# Autodesk Inventor assembly: car_2
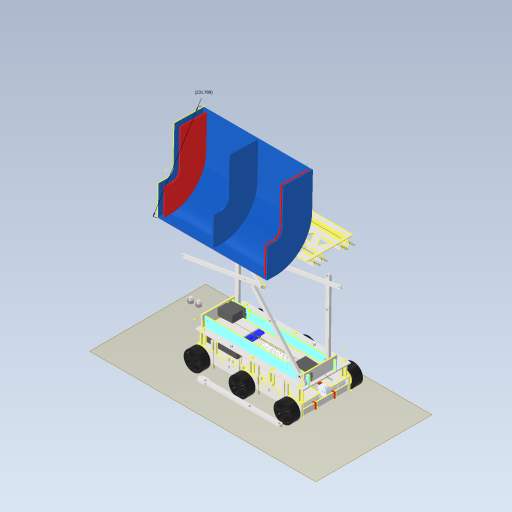
[picture p0: Inventor's stored thumbnail of the model, 512x512]
Saved by Autodesk Inventor 2023 (Build 270158000, 158)
## iProperties
Created: 2023-04-28
Part Number: car_2
Document SubType Name: Assembly
Designer: Johnny Jou
Author: Johnny Jou
## Documents named in this file (19)
- C:\Users\Johnny Jou\Documents\GitHub\Areo_Rider_Cabin\car\car_2.iam
- C:\Users\Johnny Jou\Documents\GitHub\Areo_Rider_Cabin\car\chassis_1_1_3.ipt
- C:\Users\Johnny Jou\Documents\GitHub\Areo_Rider_Cabin\car\外抓檔\25GA370.ipt
- C:\Users\Johnny Jou\Documents\GitHub\Areo_Rider_Cabin\car\chassis_1_5.ipt
- C:\Users\Johnny Jou\Documents\GitHub\Areo_Rider_Cabin\car\chassis_1_6.ipt
- C:\Users\Johnny Jou\Documents\GitHub\Areo_Rider_Cabin\car\plate_2.ipt
- C:\Users\Johnny Jou\Documents\GitHub\Areo_Rider_Cabin\car\bracket.ipt
- C:\Users\Johnny Jou\Documents\GitHub\Areo_Rider_Cabin\car\chassis_1_7.ipt
- C:\Users\Johnny Jou\Documents\GitHub\Areo_Rider_Cabin\car\bearing.ipt
- C:\Users\Johnny Jou\Documents\GitHub\Areo_Rider_Cabin\car\wheel_base_cover.ipt
- C:\Users\Johnny Jou\Documents\GitHub\Areo_Rider_Cabin\car\bracket_2.ipt
- C:\Users\Johnny Jou\Documents\GitHub\Areo_Rider_Cabin\car\外抓檔\BreadBoard.ipt
- C:\Users\Johnny Jou\Documents\GitHub\Areo_Rider_Cabin\car\外抓檔\arduino uno.ipt
- C:\Users\Johnny Jou\Documents\GitHub\Areo_Rider_Cabin\car\外抓檔\L298N.ipt
- C:\Users\Johnny Jou\Documents\GitHub\Areo_Rider_Cabin\car\外抓檔\電池和\3.7V 2X 18650 Battery Holder with On Off Switch_TOP.iam
- C:\Users\Johnny Jou\Documents\GitHub\Areo_Rider_Cabin\car\wheelsys.iam
- C:\Users\Johnny Jou\Documents\GitHub\Areo_Rider_Cabin\Expansion\test\linkage_system_test.iam
- C:\Users\Johnny Jou\Documents\GitHub\Areo_Rider_Cabin\car\axle 4_30.ipt
- C:\Users\Johnny Jou\Documents\GitHub\Areo_Rider_Cabin\Expansion\test\idler.iam
## Components (59 placed, 18 different names)
1. 25GA370:1 — 貼合:7, 貼合:9, 貼合:224
2. 25GA370:2 — 貼合:7, 貼合:8, 貼合:49, 貼合:220
3. chassis_1_5:1 — 貼合:9, 齊平:5, 齊平:10, 齊平:11, 齊平:12, 齊平:13, 貼合:13, 貼合:14, 貼合:42, 貼合:43, 貼合:51
4. chassis_1_5:2 — 貼合:8, 齊平:5, 貼合:15, 貼合:16, 貼合:17, 貼合:18, 貼合:19, 貼合:20
5. chassis_1_6:1 — 齊平:7, 齊平:8, 齊平:9, 齊平:13, 貼合:13, 貼合:14
6. chassis_1_6:2 — 齊平:8, 齊平:10, 貼合:17, 貼合:18, 貼合:42, 貼合:43, 齊平:14, 貼合:44, 貼合:45, 齊平:15
7. chassis_1_6:3 — 齊平:9, 齊平:11, 貼合:19, 貼合:20
8. chassis_1_6:4 — 齊平:7, 齊平:12, 貼合:15, 貼合:16
9. plate_2:1 — 貼合:38, 貼合:40, 貼合:41, 貼合:50, 齊平:19, 貼合:116, 齊平:25, 貼合:185, 貼合:186, 貼合:187, 貼合:188, 貼合:189, 貼合:190, 貼合:191, 貼合:192, 貼合:193, 貼合:194, 貼合:195, 貼合:196, 貼合:197, 貼合:198, 貼合:199, 貼合:200, 貼合:203, 貼合:204, 貼合:205, 貼合:206, 貼合:207, 貼合:208, 貼合:209, 貼合:210, 貼合:211
10. chassis_1_1_3:1 — 齊平:14, 貼合:44, 貼合:45, 貼合:46, 貼合:47, 貼合:48, 貼合:49, 齊平:16, 貼合:108, 貼合:110, 貼合:111, 齊平:24, 貼合:171, 貼合:172, 貼合:217, 貼合:219, 貼合:221
11. chassis_1_1_3:2 — 齊平:15, 齊平:16, 貼合:50, 齊平:19, 貼合:52, 貼合:53, 貼合:54, 貼合:55, 貼合:56, 貼合:57, 貼合:109, 齊平:24, 齊平:25, 貼合:169, 貼合:170, 貼合:223, 貼合:225, 貼合:227, 貼合:230, 貼合:231, 貼合:232, 貼合:233
12. chassis_1_7:1 — 貼合:51, 貼合:52, 貼合:53
13. chassis_1_7:2 — 貼合:54, 貼合:55, 貼合:56, 貼合:57
14. 軸承 GB/T 292-2007 類型 IN - 退回 B724 C:1 — 貼合:67, 貼合:68, 插入:2
15. wheel_base_cover:1 — 貼合:67, 貼合:68, 貼合:171, 貼合:172
16. 軸承 GB/T 292-2007 類型 IN - 退回 B724 C:2 — 插入:3
17. wheel_base_cover:2 — 貼合:108, 貼合:109
18. 軸承 GB/T 292-2007 類型 IN - 退回 B724 C:4 — 插入:1
19. wheel_base_cover:4 — 貼合:110, 貼合:111
20. bracket:10 — 貼合:116, 貼合:210
21. bracket:9 — 貼合:211
22. 軸承 GB/T 292-2007 類型 IN - 退回 B724 C:5 — 插入:4
23. wheel_base_cover:5 — 貼合:169, 貼合:170
24. bracket_2:1 — 貼合:191, 貼合:196, 貼合:197
25. bracket_2:2 — 貼合:188, 貼合:192, 貼合:193
26. bracket_2:3 — 貼合:189, 貼合:194, 貼合:198, 貼合:202
27. bracket_2:4 — 貼合:190, 貼合:195, 貼合:199
28. bracket_2:5 — 貼合:185, 貼合:186, 貼合:187, 貼合:201
29. BreadBoard:1 — 貼合:200, 貼合:201, 貼合:202
30. L298N:1 — 貼合:203, 貼合:208, 貼合:209
31. arduino uno:1 — 貼合:204, 貼合:205, 貼合:206
32. 3.7V 2X 18650 Battery Holder with On Off Switch_TOP:1 [sub-assembly] — 貼合:207
33. wheelsys:1 [sub-assembly] — 貼合:217, 相切:1
34. wheelsys:2 [sub-assembly] — 貼合:220, 貼合:221
35. wheelsys:4 [sub-assembly] — 貼合:219
36. wheelsys:5 [sub-assembly] — 貼合:227
37. wheelsys:6 [sub-assembly] — 貼合:224, 貼合:225
38. wheelsys:7 [sub-assembly] — 貼合:223
39. linkage_system_test:1 [sub-assembly] — 貼合:228, 貼合:229
40. axle 4_30:1 — 插入:1
41. axle 4_30:4 — 插入:4
42. axle 4_30:5 — 插入:3
43. axle 4_30:6 — 插入:2
44. idler:1 [sub-assembly] — 貼合:230, 貼合:231
45. idler:2 [sub-assembly] — 貼合:232, 貼合:233
46. idler:3 [sub-assembly]
47. idler:4 [sub-assembly]
48. bracket:7 — 貼合:38, 貼合:40
49. bracket:8 — 貼合:41
50. bracket:11
51. bracket:12
52. bracket:13
53. bracket:14
54. bracket:15
55. bracket:16
56. bracket:17
57. bracket:18
58. bracket:19 — 貼合:228
59. bracket:20 — 貼合:229
## Component patterns: (6 elements, first: bracket:7 + bracket:8)
## Relationships (114: Mate 94, Flush 14, Insert 4, Angle 1, Tangent 1)
- 貼合:7 [Mate] (20 mm): 25GA370:1 ↔ 25GA370:2
- 貼合:8 [Mate]: 25GA370:2 ↔ chassis_1_5:2
- 貼合:9 [Mate]: 25GA370:1 ↔ chassis_1_5:1
- 齊平:5 [Flush]: chassis_1_5:1 ↔ chassis_1_5:2
- 齊平:7 [Flush]: chassis_1_6:1 ↔ chassis_1_6:4
- 齊平:8 [Flush]: chassis_1_6:1 ↔ chassis_1_6:2
- 齊平:9 [Flush]: chassis_1_6:1 ↔ chassis_1_6:3
- 齊平:10 [Flush]: chassis_1_5:1 ↔ chassis_1_6:2
- 齊平:11 [Flush]: chassis_1_5:1 ↔ chassis_1_6:3
- 齊平:12 [Flush]: chassis_1_5:1 ↔ chassis_1_6:4
- 齊平:13 [Flush]: chassis_1_5:1 ↔ chassis_1_6:1
- 貼合:13 [Mate]: chassis_1_5:1 ↔ chassis_1_6:1
- 貼合:14 [Mate]: chassis_1_5:1 ↔ chassis_1_6:1
- 貼合:15 [Mate]: chassis_1_5:2 ↔ chassis_1_6:4
- 貼合:16 [Mate]: chassis_1_5:2 ↔ chassis_1_6:4
- 貼合:17 [Mate]: chassis_1_5:2 ↔ chassis_1_6:2
- 貼合:18 [Mate]: chassis_1_5:2 ↔ chassis_1_6:2
- 貼合:19 [Mate]: chassis_1_5:2 ↔ chassis_1_6:3
- 貼合:20 [Mate]: chassis_1_5:2 ↔ chassis_1_6:3
- [Mate]: bracket:7 ↔ bracket:8
- [Mate]: bracket:7 ↔ bracket:8
- [Mate]: bracket:7 ↔ bracket:8
- 貼合:38 [Mate]: plate_2:1 ↔ bracket:7
- 貼合:40 [Mate]: plate_2:1 ↔ bracket:7
- 貼合:41 [Mate]: plate_2:1 ↔ bracket:8
- 貼合:42 [Mate]: chassis_1_5:1 ↔ chassis_1_6:2
- 貼合:43 [Mate]: chassis_1_5:1 ↔ chassis_1_6:2
- 齊平:14 [Flush]: chassis_1_6:2 ↔ chassis_1_1_3:1
- 貼合:44 [Mate]: chassis_1_6:2 ↔ chassis_1_1_3:1
- 貼合:45 [Mate]: chassis_1_6:2 ↔ chassis_1_1_3:1
- 貼合:46 [Mate]: chassis_1_1_3:1
- 貼合:47 [Mate]: chassis_1_1_3:1
- 貼合:48 [Mate]: chassis_1_1_3:1
- 貼合:49 [Mate]: 25GA370:2 ↔ chassis_1_1_3:1
- 齊平:15 [Flush]: chassis_1_6:2 ↔ chassis_1_1_3:2
- 齊平:16 [Flush]: chassis_1_1_3:1 ↔ chassis_1_1_3:2
- 貼合:50 [Mate]: plate_2:1 ↔ chassis_1_1_3:2
- 齊平:19 [Flush]: plate_2:1 ↔ chassis_1_1_3:2
- 貼合:51 [Mate]: chassis_1_5:1 ↔ chassis_1_7:1
- 貼合:52 [Mate]: chassis_1_1_3:2 ↔ chassis_1_7:1
- 貼合:53 [Mate]: chassis_1_1_3:2 ↔ chassis_1_7:1
- 貼合:54 [Mate]: chassis_1_1_3:2 ↔ chassis_1_7:2
- 貼合:55 [Mate]: chassis_1_1_3:2 ↔ chassis_1_7:2
- 貼合:56 [Mate]: chassis_1_1_3:2 ↔ chassis_1_7:2
- 貼合:57 [Mate]: chassis_1_1_3:2 ↔ chassis_1_7:2
- 貼合:67 [Mate]: 軸承 GB/T 292-2007 類型 IN - 退回 B724 C:1 ↔ wheel_base_cover:1
- 貼合:68 [Mate]: 軸承 GB/T 292-2007 類型 IN - 退回 B724 C:1 ↔ wheel_base_cover:1
- [Mate]: 軸承 GB/T 292-2007 類型 IN - 退回 B724 C:2 ↔ wheel_base_cover:2
- [Mate]: 軸承 GB/T 292-2007 類型 IN - 退回 B724 C:2 ↔ wheel_base_cover:2
- [Mate]: 軸承 GB/T 292-2007 類型 IN - 退回 B724 C:4 ↔ wheel_base_cover:4
- [Mate]: 軸承 GB/T 292-2007 類型 IN - 退回 B724 C:4 ↔ wheel_base_cover:4
- 貼合:108 [Mate]: chassis_1_1_3:1 ↔ wheel_base_cover:2
- 貼合:109 [Mate]: chassis_1_1_3:2 ↔ wheel_base_cover:2
- 貼合:110 [Mate]: chassis_1_1_3:1 ↔ wheel_base_cover:4
- 貼合:111 [Mate]: chassis_1_1_3:1 ↔ wheel_base_cover:4
- [Mate]: bracket:10 ↔ bracket:9
- [Mate]: bracket:10 ↔ bracket:9
- [Mate]: bracket:10 ↔ bracket:9
- 貼合:116 [Mate]: plate_2:1 ↔ bracket:10
- 齊平:24 [Flush]: chassis_1_1_3:1 ↔ chassis_1_1_3:2
- 齊平:25 [Flush]: plate_2:1 ↔ chassis_1_1_3:2
- [Mate]: 軸承 GB/T 292-2007 類型 IN - 退回 B724 C:5 ↔ wheel_base_cover:5
- [Mate]: 軸承 GB/T 292-2007 類型 IN - 退回 B724 C:5 ↔ wheel_base_cover:5
- 貼合:169 [Mate]: chassis_1_1_3:2 ↔ wheel_base_cover:5
- 貼合:170 [Mate]: chassis_1_1_3:2 ↔ wheel_base_cover:5
- 貼合:171 [Mate]: chassis_1_1_3:1 ↔ wheel_base_cover:1
- 貼合:172 [Mate]: chassis_1_1_3:1 ↔ wheel_base_cover:1
- 貼合:185 [Mate]: plate_2:1 ↔ bracket_2:5
- 貼合:186 [Mate]: plate_2:1 ↔ bracket_2:5
- 貼合:187 [Mate]: plate_2:1 ↔ bracket_2:5
- 貼合:188 [Mate]: plate_2:1 ↔ bracket_2:2
- 貼合:189 [Mate]: plate_2:1 ↔ bracket_2:3
- 貼合:190 [Mate]: plate_2:1 ↔ bracket_2:4
- 貼合:191 [Mate]: plate_2:1 ↔ bracket_2:1
- 貼合:192 [Mate]: plate_2:1 ↔ bracket_2:2
- 貼合:193 [Mate]: plate_2:1 ↔ bracket_2:2
- 貼合:194 [Mate]: plate_2:1 ↔ bracket_2:3
- 貼合:195 [Mate]: plate_2:1 ↔ bracket_2:4
- 貼合:196 [Mate]: plate_2:1 ↔ bracket_2:1
- 貼合:197 [Mate]: plate_2:1 ↔ bracket_2:1
- 貼合:198 [Mate]: plate_2:1 ↔ bracket_2:3
- 貼合:199 [Mate]: plate_2:1 ↔ bracket_2:4
- 貼合:200 [Mate]: plate_2:1 ↔ BreadBoard:1
- 貼合:201 [Mate]: bracket_2:5 ↔ BreadBoard:1
- 貼合:202 [Mate]: bracket_2:3 ↔ BreadBoard:1
- 貼合:203 [Mate]: plate_2:1 ↔ L298N:1
- 貼合:204 [Mate] (2 mm): plate_2:1 ↔ arduino uno:1
- 貼合:205 [Mate]: plate_2:1 ↔ arduino uno:1
- 貼合:206 [Mate]: plate_2:1 ↔ arduino uno:1
- 貼合:207 [Mate]: plate_2:1 ↔ 3.7V 2X 18650 Battery Holder with On Off Switch_TOP:1
- 貼合:208 [Mate]: plate_2:1 ↔ L298N:1
- 貼合:209 [Mate]: plate_2:1 ↔ L298N:1
- 貼合:210 [Mate]: plate_2:1 ↔ bracket:10
- 貼合:211 [Mate]: plate_2:1 ↔ bracket:9
- 貼合:217 [Mate] (1 mm): chassis_1_1_3:1 ↔ wheelsys:1
- 貼合:219 [Mate] (1 mm): chassis_1_1_3:1 ↔ wheelsys:4
- 貼合:220 [Mate]: 25GA370:2 ↔ wheelsys:2
- 貼合:221 [Mate] (1 mm): chassis_1_1_3:1 ↔ wheelsys:2
- 貼合:223 [Mate] (1 mm): chassis_1_1_3:2 ↔ wheelsys:7
- 貼合:224 [Mate]: 25GA370:1 ↔ wheelsys:6
- 貼合:225 [Mate] (1 mm): chassis_1_1_3:2 ↔ wheelsys:6
- 貼合:227 [Mate] (1 mm): chassis_1_1_3:2 ↔ wheelsys:5
- 貼合:228 [Mate]: linkage_system_test:1 ↔ bracket:19
- 貼合:229 [Mate]: linkage_system_test:1 ↔ bracket:20
- 角度:1 [Angle] (0 deg)
- 相切:1 [Tangent]: wheelsys:1
- 插入:1 [Insert]: 軸承 GB/T 292-2007 類型 IN - 退回 B724 C:4 ↔ axle 4_30:1
- 插入:2 [Insert]: 軸承 GB/T 292-2007 類型 IN - 退回 B724 C:1 ↔ axle 4_30:6
- 插入:3 [Insert]: 軸承 GB/T 292-2007 類型 IN - 退回 B724 C:2 ↔ axle 4_30:5
- 插入:4 [Insert]: 軸承 GB/T 292-2007 類型 IN - 退回 B724 C:5 ↔ axle 4_30:4
- 貼合:230 [Mate]: chassis_1_1_3:2 ↔ idler:1
- 貼合:231 [Mate]: chassis_1_1_3:2 ↔ idler:1
- 貼合:232 [Mate]: chassis_1_1_3:2 ↔ idler:2
- 貼合:233 [Mate]: chassis_1_1_3:2 ↔ idler:2
## Named parameters: d54_d45 = 0 mm, d55_d46 = 0 mm, d56_d47 = 0 mm, d121_d107 = 0 mm, d122_d108 = 0 mm, d147_d107 = 0 mm, d148_d108 = 0 mm, d209_d54_d45 = 0 mm, d210_d55_d46 = 0 mm, d211_d56_d47 = 0 mm, d233_d107 = 0 mm, d234_d108 = 0 mm
